# Autodesk Inventor assembly: Fan_Assembled
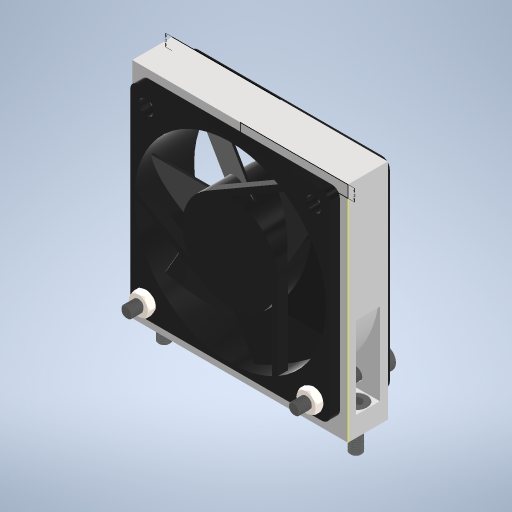
[picture p0: Inventor's stored thumbnail of the model, 512x512]
Saved by Autodesk Inventor 2023.1 (Build 271208000, 208)
## iProperties
Created: 2023-12-08
Part Number: Fan_Assembled
Document SubType Name: Assembly
Designer: JansenL
Author: JansenL
## Documents named in this file (6)
- C:\Users\JansenL\Documents\FHM\Semester_1\ProjektMech\CAD-files\Fan_Assembled.iam
- C:\Users\JansenL\Documents\FHM\Semester_1\ProjektMech\CAD-files\FAN\Fan.ipt
- C:\Users\JansenL\Documents\FHM\Semester_1\ProjektMech\CAD-files\Aufnahme_Fan_02.ipt
- C:\Users\JansenL\Documents\FHM\Semester_1\ProjektMech\CAD-files\M3_Screws\M3x20.ipt
- C:\Users\JansenL\Documents\FHM\Semester_1\ProjektMech\CAD-files\M3_Screws\M3_Nut.ipt
- C:\Users\JansenL\Documents\FHM\Semester_1\ProjektMech\CAD-files\M3_Screws\M3x10.ipt
## Components (9 placed, 5 different names)
1. Fan:1 — Mate:4, Mate:5, Mate:6, Mate:7, Mate:8, Mate:9, Mate:10, Mate:11, Mate:12, Mate:13, Mate:14, Mate:18, Mate:19
2. Aufnahme_Fan_02:1 — Mate:6, Mate:7, Mate:8, Mate:20, Mate:23
3. Aufnahme_Fan_02:2 — Mate:9, Mate:10, Mate:11, Mate:15, Mate:21, Mate:22
4. M3x20:1 — Mate:13, Mate:16
5. M3x20:2 — Mate:12, Mate:14, Mate:17
6. M3_Nut:1 — Mate:17, Mate:19
7. M3_Nut:2 — Mate:16, Mate:18
8. M3x10:1 — Mate:20, Mate:23
9. M3x10:2 — Mate:21, Mate:22
## Relationships (20: Mate 20)
- Mate:4: Fan:1
- Mate:5: Fan:1
- Mate:6: Fan:1 ↔ Aufnahme_Fan_02:1
- Mate:7: Fan:1 ↔ Aufnahme_Fan_02:1
- Mate:8: Fan:1 ↔ Aufnahme_Fan_02:1
- Mate:9: Fan:1 ↔ Aufnahme_Fan_02:2
- Mate:10: Fan:1 ↔ Aufnahme_Fan_02:2
- Mate:11: Fan:1 ↔ Aufnahme_Fan_02:2
- Mate:12: Fan:1 ↔ M3x20:2
- Mate:13: Fan:1 ↔ M3x20:1
- Mate:14: Fan:1 ↔ M3x20:2
- Mate:15: Aufnahme_Fan_02:2
- Mate:16: M3x20:1 ↔ M3_Nut:2
- Mate:17: M3x20:2 ↔ M3_Nut:1
- Mate:18: Fan:1 ↔ M3_Nut:2
- Mate:19: Fan:1 ↔ M3_Nut:1
- Mate:20: Aufnahme_Fan_02:1 ↔ M3x10:1
- Mate:21: Aufnahme_Fan_02:2 ↔ M3x10:2
- Mate:22: Aufnahme_Fan_02:2 ↔ M3x10:2
- Mate:23: Aufnahme_Fan_02:1 ↔ M3x10:1
